# Autodesk Inventor assembly: 7in Display Module
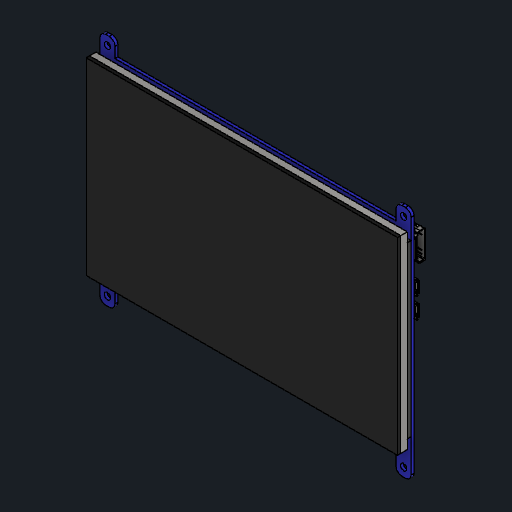
[picture p0: Inventor's stored thumbnail of the model, 512x512]
Saved by Autodesk Inventor 2026.2 (Build 302298000, 298)
## iProperties
Created: 2026-01-24
Part Number: 7in Display Module
Document SubType Name: Assembly
Designer: JoshuaEah
Author: JoshuaEah
## Documents named in this file (4)
- C:\Users\JoshuaEah\Documents\GitHub\Voron-0\CAD\Display\Parts\7in Display Module.iam
- C:\Users\JoshuaEah\Documents\GitHub\Voron-0\CAD\Display\Parts\7in Touch Display.ipt
- C:\Users\JoshuaEah\Documents\GitHub\Voron-0\CAD\Display\Parts\HDMI Connector.ipt
- C:\Users\JoshuaEah\Documents\GitHub\Voron-0\CAD\Display\Parts\USB Micro-B.ipt
## Components (4 placed, 3 different names)
1. 7in Touch Display:1 — Flush:1, Flush:2, Mate:1, Mate:3, Flush:3, Flush:4, Mate:4
2. HDMI Connector:1 — Flush:1, Flush:2, Mate:1, Mate:2
3. USB Micro-B:1 — Mate:2, Mate:3, Flush:3, Mate:5
4. USB Micro-B:2 — Flush:4, Mate:4, Mate:5
## Relationships (9: Mate 5, Flush 4)
- Flush:1 (11.4 mm): 7in Touch Display:1 ↔ HDMI Connector:1
- Flush:2: 7in Touch Display:1 ↔ HDMI Connector:1
- Mate:1 (0.635 mm): 7in Touch Display:1 ↔ HDMI Connector:1
- Mate:2 (7 mm): HDMI Connector:1 ↔ USB Micro-B:1
- Mate:3 (0.325 mm): 7in Touch Display:1 ↔ USB Micro-B:1
- Flush:3 (0.53 mm): 7in Touch Display:1 ↔ USB Micro-B:1
- Flush:4 (0.53 mm): 7in Touch Display:1 ↔ USB Micro-B:2
- Mate:4 (0.325 mm): 7in Touch Display:1 ↔ USB Micro-B:2
- Mate:5 (3.5 mm): USB Micro-B:1 ↔ USB Micro-B:2
